# Autodesk Inventor assembly: omniwheel_MIR
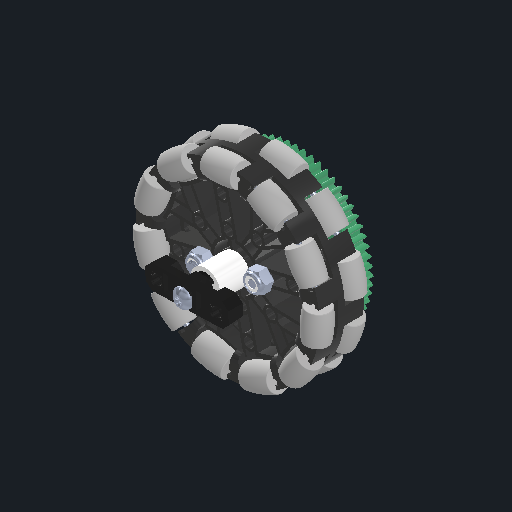
[picture p0: Inventor's stored thumbnail of the model, 512x512]
Saved by Autodesk Inventor 2024 (Build 280153000, 153)
## iProperties
Created: 2023-08-09
Part Number: omniwheel_MIR
Document SubType Name: Assembly
Designer: macbook
Author: macbook
## Documents named in this file (19)
- \\Mac\Home\Desktop\code\1599V-VRC\Cad\Assembly\v2\omniwheel_MIR.iam
- \\Mac\Home\Desktop\code\1599V-VRC\Cad\Motion\Wheels\Omni Wheel\3.25 Omni AS, cir_MIR.iam
- \\Mac\Home\Desktop\code\1599V-VRC\Cad\Motion\Spacers\Spacer Nylon Click On\Nspacer Click On x .1250.ipt
- \\Mac\Home\Desktop\code\1599V-VRC\Cad\Motion\Spacers\Spacer Nylon Click On.ipt
- \\Mac\Home\Desktop\code\1599V-VRC\Cad\Motion\Shaft LS\Bearing Flat_MIR5.ipt
- \\Mac\Home\Desktop\code\1599V-VRC\Cad\Motion\Gears\LS 60T Gear_MIR3.ipt
- \\Mac\Home\Desktop\code\1599V-VRC\Cad\Structure\Hardware\Screw Steel - Star\SScrew Star Threaded 1.250.ipt
- \\Mac\Home\Desktop\code\1599V-VRC\Cad\Structure\Hardware\Screw Steel - Star.ipt
- \\Mac\Home\Desktop\code\1599V-VRC\Cad\Structure\Hardware\Nut Nylock_MIR5.ipt
- \\Mac\Home\Desktop\code\1599V-VRC\Cad\Structure\Hardware\Screw Steel - Star\SScrew Star Smooth 2.500.ipt
- \\Mac\Home\Desktop\code\1599V-VRC\Cad\Structure\C Channel\Aluminum 1x2x1\Alu C 1x2x1x14_MIR2.ipt
- \\Mac\Home\Desktop\code\1599V-VRC\Cad\Motion\Spacers\Spacer Nylon .500 OD\NSpacer White .500 OD x .500.ipt
- \\Mac\Home\Desktop\code\1599V-VRC\Cad\Motion\Spacers\Spacer Nylon .500 OD.ipt
- \\Mac\Home\Desktop\code\1599V-VRC\Cad\Motion\Spacers\Washer Steel\SWasher .375 OD x .015625.ipt
- \\Mac\Home\Desktop\code\1599V-VRC\Cad\Motion\Spacers\Washer Steel.ipt
- \\Mac\Home\Desktop\code\1599V-VRC\Cad\Motion\Spacers\Spacer Nylon .500 OD\NSpacer White .500 OD x .375.ipt
- \\Mac\Home\Desktop\code\1599V-VRC\Cad\Motion\Spacers\Washer Teflon\TWasher .375 OD x .03125.ipt
- \\Mac\Home\Desktop\code\1599V-VRC\Cad\Motion\Spacers\Washer Teflon.ipt
- \\Mac\Home\Desktop\code\1599V-VRC\Cad\Motion\Spacers\Spacer Nylon Click On\Nspacer Click On x .0625.ipt
## Components (19 placed, 13 different names)
1. 3.25 Omni AS, cir_MIR:1 [sub-assembly] — Insert:97, Insert:95, Insert:94, Insert:92
2. Nspacer Click On x .1250:1 — Insert:98
3. Bearing Flat_MIR5:1 — Insert:47, Insert:46, Insert:71
4. Bearing Flat_MIR5:2 — Insert:47, Insert:46, Insert:70, Insert:73, Insert:72, Insert:99
5. LS 60T Gear_MIR3:1 — Insert:82, Insert:84, Insert:86, Insert:91, Insert:98
6. SScrew Star Threaded 1.250:1 — Insert:83, Rotational:1
7. Nut Nylock_MIR5:1 — Insert:94, Rotational:1
8. Nut Nylock_MIR5:2 — Insert:97
9. SScrew Star Threaded 1.250:2 — Insert:85
10. SScrew Star Smooth 2.500:3 — Insert:70
11. Nut Nylock_MIR5:3 — Insert:71
12. Alu C 1x2x1x14_MIR2:1 — Insert:73, Insert:72
13. NSpacer White .500 OD x .500:1 — Insert:95, Insert:96
14. SWasher .375 OD x .015625:1 — Insert:82, Insert:81
15. NSpacer White .500 OD x .375:2 — Insert:81
16. TWasher .375 OD x .03125:1 — Insert:84, Insert:83
17. TWasher .375 OD x .03125:2 — Insert:86, Insert:85
18. Nspacer Click On x .0625:2 — Insert:99, Insert:96
19. NSpacer White .500 OD x .375:3 — Insert:91, Insert:92
## Relationships (21: Insert 20, RevoluteJoint 1)
- Insert:47 (44.45 mm): Bearing Flat_MIR5:1 ↔ Bearing Flat_MIR5:2
- Insert:46 (44.45 mm): Bearing Flat_MIR5:1 ↔ Bearing Flat_MIR5:2
- Insert:70 (1.5875 mm): Bearing Flat_MIR5:2 ↔ SScrew Star Smooth 2.500:3
- Insert:71: Bearing Flat_MIR5:1 ↔ Nut Nylock_MIR5:3
- Insert:73: Bearing Flat_MIR5:2 ↔ Alu C 1x2x1x14_MIR2:1
- Insert:72: Bearing Flat_MIR5:2 ↔ Alu C 1x2x1x14_MIR2:1
- Insert:82: LS 60T Gear_MIR3:1 ↔ SWasher .375 OD x .015625:1
- Insert:81: SWasher .375 OD x .015625:1 ↔ NSpacer White .500 OD x .375:2
- Insert:84: LS 60T Gear_MIR3:1 ↔ TWasher .375 OD x .03125:1
- Insert:83: SScrew Star Threaded 1.250:1 ↔ TWasher .375 OD x .03125:1
- Insert:86: LS 60T Gear_MIR3:1 ↔ TWasher .375 OD x .03125:2
- Insert:85: SScrew Star Threaded 1.250:2 ↔ TWasher .375 OD x .03125:2
- Insert:91: LS 60T Gear_MIR3:1 ↔ NSpacer White .500 OD x .375:3
- Insert:98: Nspacer Click On x .1250:1 ↔ LS 60T Gear_MIR3:1
- Insert:97: 3.25 Omni AS, cir_MIR:1 ↔ Nut Nylock_MIR5:2
- Insert:95: 3.25 Omni AS, cir_MIR:1 ↔ NSpacer White .500 OD x .500:1
- Insert:94: 3.25 Omni AS, cir_MIR:1 ↔ Nut Nylock_MIR5:1
- Insert:92: 3.25 Omni AS, cir_MIR:1 ↔ NSpacer White .500 OD x .375:3
- Insert:99: Bearing Flat_MIR5:2 ↔ Nspacer Click On x .0625:2
- Insert:96: NSpacer White .500 OD x .500:1 ↔ Nspacer Click On x .0625:2
- Rotational:1 [RevoluteJoint]: SScrew Star Threaded 1.250:1 ↔ Nut Nylock_MIR5:1
